# Autodesk Inventor assembly: Крепление мотора
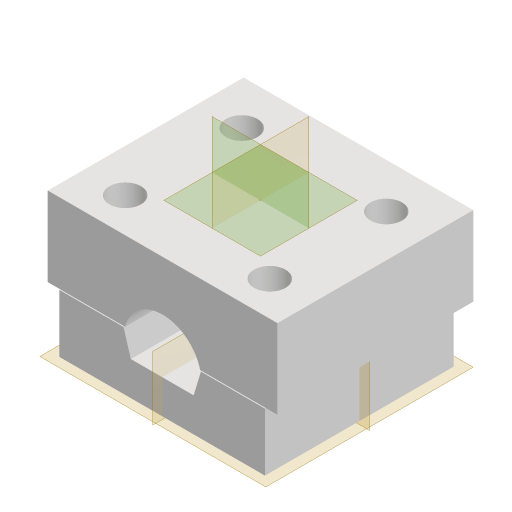
[picture p0: Inventor's stored thumbnail of the model, 512x512]
Saved by Autodesk Inventor 2023.2 (Build 272271030, 271C)
## iProperties
Created: 2024-12-18
Part Number: Крепление мотора
Document SubType Name: Assembly
Designer: I9232
Author: I9232
## Documents named in this file (3)
- D:\!Cheburashka\Cheburashka_construction\Rover\Крепление мотора.iam
- D:\!Cheburashka\Cheburashka_construction\Rover\Крепление мотора.ipt
- D:\!Cheburashka\Cheburashka_construction\Rover\Крепление мотора2.ipt
## Components (2 placed, 2 different names)
1. Нижняя часть крепления мотора:1 — Совмещение:1, Совмещение:2
2. Крепление мотора2:1 — Совмещение:1, Совмещение:2
## Relationships (2: Mate 2)
- Совмещение:1 [Mate]: Нижняя часть крепления мотора:1 ↔ Крепление мотора2:1
- Совмещение:2 [Mate]: Нижняя часть крепления мотора:1 ↔ Крепление мотора2:1
